# Autodesk Inventor assembly: SA-117_v0.1
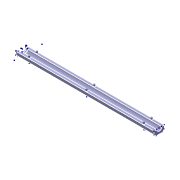
[picture p0: Inventor's stored thumbnail of the model, 180x180]
Saved by Autodesk Inventor 2017 (Build 210142000, 142)
## iProperties
Created: 2018-10-11
Part Number: SA-117_v0.1
Document SubType Name: Assembly
Designer: Kathryn Rosie
Author: Kathryn Rosie
## Documents named in this file (3)
- C:\Users\Kathryn Rosie\Google Drive\HERA\Feed\CAD\SA-117_v0.1.iam
- C:\Users\Kathryn Rosie\Google Drive\HERA\Feed\CAD\Dan 20181009 SA117\DP-116_v0.1_Rev_A.ipt
- C:\Users\Kathryn Rosie\Google Drive\HERA\Feed\CAD\DP-115A_v0.1.ipt
## Components (7 placed, 2 different names)
1. DP-115A_v0.1:1 — Mate:1, Mate:2, Mate:3, Mate:4, Mate:5, Mate:6, Mate:7, Mate:8, Mate:9, Mate:10, Mate:11, Mate:12
2. DP-116_v0.1_Rev_A:1 — Mate:1, Mate:8
3. DP-116_v0.1_Rev_A:2 — Mate:2, Mate:9
4. DP-116_v0.1_Rev_A:3 — Mate:3, Mate:11
5. DP-116_v0.1_Rev_A:4 — Mate:4, Mate:12
6. DP-116_v0.1_Rev_A:5 — Mate:5, Mate:10
7. DP-116_v0.1_Rev_A:6 — Mate:6, Mate:7
## Relationships (12: Mate 12)
- Mate:1: DP-115A_v0.1:1 ↔ DP-116_v0.1_Rev_A:1
- Mate:2: DP-115A_v0.1:1 ↔ DP-116_v0.1_Rev_A:2
- Mate:3: DP-115A_v0.1:1 ↔ DP-116_v0.1_Rev_A:3
- Mate:4: DP-115A_v0.1:1 ↔ DP-116_v0.1_Rev_A:4
- Mate:5: DP-115A_v0.1:1 ↔ DP-116_v0.1_Rev_A:5
- Mate:6: DP-115A_v0.1:1 ↔ DP-116_v0.1_Rev_A:6
- Mate:7 (-7 mm): DP-115A_v0.1:1 ↔ DP-116_v0.1_Rev_A:6
- Mate:8 (-7 mm): DP-115A_v0.1:1 ↔ DP-116_v0.1_Rev_A:1
- Mate:9 (-7 mm): DP-115A_v0.1:1 ↔ DP-116_v0.1_Rev_A:2
- Mate:10 (-7 mm): DP-115A_v0.1:1 ↔ DP-116_v0.1_Rev_A:5
- Mate:11 (-7 mm): DP-115A_v0.1:1 ↔ DP-116_v0.1_Rev_A:3
- Mate:12 (-7 mm): DP-115A_v0.1:1 ↔ DP-116_v0.1_Rev_A:4
